# Autodesk Inventor assembly: all-the-parts
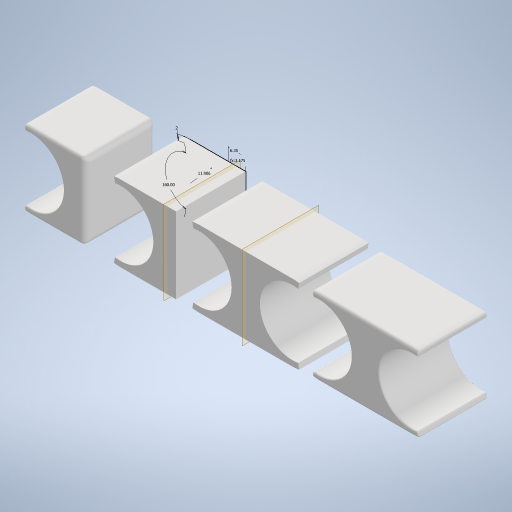
[picture p0: Inventor's stored thumbnail of the model, 512x512]
Saved by Autodesk Inventor 2023.1 (Build 271208000, 208)
## iProperties
Created: 2023-03-31
Part Number: all-the-parts
Document SubType Name: Assembly
Designer: caleb
Author: caleb
## Documents named in this file (5)
- N:\caleb\laser\kevin\kevin-hook-thingy\all-the-parts.iam
- N:\caleb\laser\kevin\kevin-hook-thingy\base-fileted.ipt
- N:\caleb\laser\kevin\kevin-hook-thingy\hook-thingy-base.ipt
- N:\caleb\laser\kevin\kevin-hook-thingy\two-sided.ipt
- N:\caleb\laser\kevin\kevin-hook-thingy\two-sided-fillet.ipt
## Components (4 placed, 4 different names)
1. base-fileted:1 — Flush:1, Flush:6
2. hook-thingy-base:1 — Flush:1, Flush:2, Flush:5, Flush:6
3. two-sided:1 — Flush:2, Flush:3, Flush:4, Flush:5
4. two-sided-fillet:1 — Flush:3, Flush:4
## Relationships (6: Flush 6)
- Flush:1: base-fileted:1 ↔ hook-thingy-base:1
- Flush:2: hook-thingy-base:1 ↔ two-sided:1
- Flush:3: two-sided:1 ↔ two-sided-fillet:1
- Flush:4: two-sided:1 ↔ two-sided-fillet:1
- Flush:5: hook-thingy-base:1 ↔ two-sided:1
- Flush:6: base-fileted:1 ↔ hook-thingy-base:1
